# Autodesk Inventor assembly: Assembly2
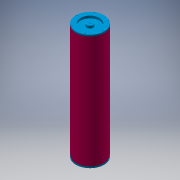
[picture p0: Inventor's stored thumbnail of the model, 180x180]
Saved by Autodesk Inventor 2016 (Build 200138000, 138)
## iProperties
Created: 2017-01-31
Part Number: Assembly2
Document SubType Name: Assembly
Designer: Student
Author: Student
## Documents named in this file (3)
- D:\junior\Assembly2.iam
- C:\Users\Student\Desktop\O ring Plug 1.ipt
- C:\Users\Student\Desktop\Noah Code\4 inch PVC pipe.ipt
## Components (3 placed, 2 different names)
1. O ring Plug 1:2 — Mate:1
2. 4 inch PVC pipe:1 — Mate:1, Mate:2
3. O ring Plug 1:3 — Mate:2
## Relationships (2: Mate 2)
- Mate:1: O ring Plug 1:2 ↔ 4 inch PVC pipe:1
- Mate:2: 4 inch PVC pipe:1 ↔ O ring Plug 1:3
